# Autodesk Inventor assembly: SAFRS-L-0001
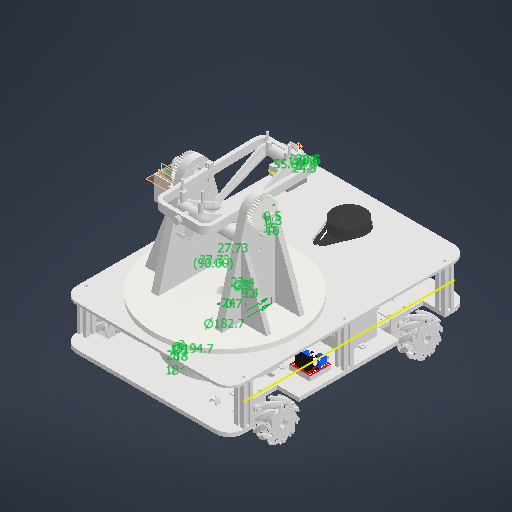
[picture p0: Inventor's stored thumbnail of the model, 512x512]
Saved by Autodesk Inventor 2026.2 (Build 302298000, 298)
## iProperties
Created: 2025-11-28
Part Number: SAFRS-L-0001
Document SubType Name: Assembly
Designer: jaewook
Author: jaewook
Title: SAFRS AGV Aseembly
## Documents named in this file (39)
- C:\Users\jk000\OneDrive\Desktop\git\SAFRS\mechanical\SAFRS_export\safrs_agv_assembly.iam
- C:\Users\jk000\OneDrive\Desktop\git\SAFRS\mechanical\SAFRS_export\01_parts\lower_plate.ipt
- C:\Users\jk000\OneDrive\Desktop\git\SAFRS\mechanical\SAFRS_export\01_parts\profile.ipt
- C:\Users\jk000\OneDrive\Desktop\git\SAFRS\mechanical\inventor\02_subassemblies\arduino_mega.iam
- C:\Users\jk000\OneDrive\Desktop\git\SAFRS\mechanical\inventor\02_subassemblies\stm32_assembly.iam
- C:\Users\jk000\OneDrive\Desktop\git\SAFRS\mechanical\inventor\02_subassemblies\L298N_motor_driver.iam
- C:\Users\jk000\OneDrive\Desktop\git\SAFRS\mechanical\SAFRS_export\01_parts\motor_connector.ipt
- C:\Users\jk000\OneDrive\Desktop\git\SAFRS\mechanical\SAFRS_export\01_parts\jgb37_520_motor_12v_319rpm.ipt
- C:\Users\jk000\OneDrive\Desktop\git\SAFRS\mechanical\inventor\02_subassemblies\dc_converter.iam
- C:\Users\jk000\OneDrive\Desktop\git\SAFRS\mechanical\SAFRS_export\01_parts\upper_plate.ipt
- C:\Users\jk000\OneDrive\Desktop\git\SAFRS\mechanical\inventor\02_subassemblies\yaw_motor_mount.iam
- C:\Users\jk000\OneDrive\Desktop\git\SAFRS\mechanical\SAFRS_export\01_parts\connector.ipt
- C:\Users\jk000\OneDrive\Desktop\git\SAFRS\mechanical\SAFRS_export\01_parts\carrier_v2.ipt
- C:\Users\jk000\OneDrive\Desktop\git\SAFRS\mechanical\SAFRS_export\01_parts\gear_support.ipt
- C:\Users\jk000\OneDrive\Desktop\git\SAFRS\mechanical\SAFRS_export\01_parts\spur_gear_15t.ipt
- C:\Users\jk000\OneDrive\Desktop\git\SAFRS\mechanical\SAFRS_export\01_parts\spur_gear_26t.ipt
- C:\Users\jk000\OneDrive\Desktop\git\SAFRS\mechanical\SAFRS_export\01_parts\spur_gear_13t.ipt
- C:\Users\jk000\OneDrive\Desktop\git\SAFRS\mechanical\SAFRS_export\01_parts\pitch_axis.ipt
- C:\Users\jk000\OneDrive\Desktop\git\SAFRS\mechanical\SAFRS_export\01_parts\pitch_axis_opposite.ipt
- C:\Users\jk000\OneDrive\Desktop\git\SAFRS\mechanical\SAFRS_export\01_parts\custom_bearing.ipt
- C:\Users\jk000\OneDrive\Desktop\git\SAFRS\mechanical\SAFRS_export\01_parts\spur_gear_22t.ipt
- C:\Users\jk000\OneDrive\Desktop\git\SAFRS\mechanical\SAFRS_export\01_parts\spur_gear_12t.ipt
- C:\Users\jk000\OneDrive\Desktop\git\SAFRS\mechanical\SAFRS_export\01_parts\pitch_motor.ipt
- C:\Users\jk000\OneDrive\Desktop\git\SAFRS\mechanical\inventor\02_subassemblies\roll_support_front_v2.iam
- C:\Users\jk000\OneDrive\Desktop\git\SAFRS\mechanical\inventor\02_subassemblies\roll_support_left_v1.iam
- C:\Users\jk000\OneDrive\Desktop\git\SAFRS\mechanical\inventor\02_subassemblies\roll_support_right.iam
- C:\Users\jk000\OneDrive\Desktop\git\SAFRS\mechanical\SAFRS_export\01_parts\key_v2.ipt
- C:\Users\jk000\OneDrive\Desktop\git\SAFRS\mechanical\SAFRS_export\01_parts\support_25mm.ipt
- C:\Users\jk000\OneDrive\Desktop\git\SAFRS\mechanical\inventor\02_subassemblies\fixer_assembly.iam
- C:\Users\jk000\OneDrive\Desktop\git\SAFRS\mechanical\SAFRS_export\01_parts\screw_v1.ipt
- C:\Users\jk000\OneDrive\Desktop\git\SAFRS\mechanical\inventor\02_subassemblies\lidar_base.iam
- C:\Users\jk000\OneDrive\Desktop\git\SAFRS\mechanical\SAFRS_export\01_parts\thrust_bearing_v1.ipt
- C:\Users\jk000\OneDrive\Desktop\git\SAFRS\mechanical\SAFRS_export\01_parts\short_screw.ipt
- C:\Users\jk000\OneDrive\Desktop\git\SAFRS\mechanical\SAFRS_export\01_parts\mecanum_wheel_75mm_left.ipt
- C:\Users\jk000\OneDrive\Desktop\git\SAFRS\mechanical\inventor\02_subassemblies\roll_support_rear_v1.iam
- C:\Users\jk000\OneDrive\Desktop\git\SAFRS\mechanical\inventor\02_subassemblies\battery_pack_mir.iam
- C:\Users\jk000\OneDrive\Desktop\git\SAFRS\mechanical\SAFRS_export\01_parts\pin.ipt
- C:\Users\jk000\OneDrive\Desktop\git\SAFRS\mechanical\SAFRS_export\01_parts\spur_gear_22t_opposite.ipt
- C:\Users\jk000\OneDrive\Desktop\git\SAFRS\mechanical\SAFRS_export\01_parts\Wire_aisle_v1.ipt
## Components (68 placed, 35 different names)
1. lower_plate:1 — 강체:1, 강체:2, 강체:3, 강체:4, 강체:5, 강체:6, 회전:1, 회전:2, 강체:8, 강체:9, 강체:10, 회전:3, 회전:4, 회전:5, 강체:11, 메이트:1, 메이트:2, 메이트:3, 메이트:6, 메이트:7, 메이트:9, 메이트:10, 메이트:18, 메이트:66, 메이트:67, 메이트:68, 메이트:69, 메이트:70, 메이트:71, 메이트:91, 메이트:92
2. profile:1 — 강체:1, 메이트:4
3. profile:2 — 강체:2
4. profile:3 — 강체:3, 메이트:5
5. profile:4 — 강체:4
6. profile:5 — 강체:5
7. profile:6 — 강체:6
8. arduino_mega:1 [sub-assembly] — 회전:1
9. stm32_assembly:1 [sub-assembly] — 회전:2
10. L298N_motor_driver:1 [sub-assembly] — 강체:8
11. L298N_motor_driver:2 [sub-assembly] — 강체:9
12. motor_connector:2 — 강체:10, 회전:9
13. motor_connector:3 — 회전:3, 회전:8
14. motor_connector:4 — 회전:4, 회전:7
15. motor_connector:5 — 회전:5, 회전:6
16. jgb37_520_motor_12v_319rpm:1 — 회전:6, 메이트:72, 메이트:73
17. jgb37_520_motor_12v_319rpm:2 — 회전:7, 메이트:74, 메이트:75
18. jgb37_520_motor_12v_319rpm:3 — 회전:8, 메이트:78, 메이트:79
19. jgb37_520_motor_12v_319rpm:4 — 회전:9, 메이트:76, 메이트:77
20. dc_converter:1 [sub-assembly] — 강체:11
21. dc_converter:2 [sub-assembly] — 메이트:1, 메이트:2, 메이트:3
22. upper_plate:1 — 메이트:4, 메이트:5, 메이트:89, 메이트:90, 메이트:93, 메이트:94, 메이트:95
23. yaw_motor_mount:1 [sub-assembly] — 메이트:6, 메이트:7, 메이트:8, 메이트:14
24. connector:1 — 메이트:8, 메이트:11, 메이트:12, 메이트:14, 메이트:15, 메이트:24
25. carrier_v2:1 — 메이트:9, 메이트:10, 메이트:18, 메이트:19, 메이트:20, 메이트:21, 메이트:22, 메이트:23, 플러쉬:1, 메이트:104, 메이트:105
26. gear_support:2 — 메이트:11, 메이트:12, 메이트:15, 메이트:16, 메이트:17
27. 스퍼 기어1:1 — 메이트:16, 메이트:17
28. 스퍼 기어2:1 — 메이트:19, 메이트:22
29. 스퍼 기어2:2 — 메이트:20, 메이트:23, 플러쉬:2
30. 스퍼 기어2:3 — 메이트:21, 플러쉬:1
31. 스퍼 기어1:2 — 메이트:24, 플러쉬:2, 메이트:25, 메이트:26, 메이트:27, 메이트:28, 메이트:29, 메이트:30
32. pitch_axis:1 — 메이트:25, 메이트:26, 메이트:27, 메이트:31, 메이트:32, 메이트:35, 메이트:37, 메이트:38, 메이트:44, 메이트:45
33. pitch_axis_opposite:1 — 메이트:28, 메이트:29, 메이트:30, 메이트:33, 메이트:34, 메이트:99
34. custom_bearing:1 — 메이트:31, 메이트:32, 메이트:36
35. custom_bearing:2 — 메이트:33, 메이트:34
36. 스퍼 기어2:4 — 메이트:35, 메이트:36, 메이트:59, 메이트:103
37. 스퍼 기어1:3 — 메이트:37, 메이트:38, 메이트:39, 메이트:40, 메이트:41
38. pitch_motor:1 — 메이트:39, 메이트:40, 메이트:41
39. pitch_motor:2 — 메이트:44, 메이트:45
40. roll_support_front_v2:1 [sub-assembly] — 메이트:52, 메이트:96, 강체:12
41. roll_support_rear_v1:1 [sub-assembly] — 메이트:97, 강체:13, 메이트:98, 메이트:100, 메이트:102
42. roll_support_left_v1:1 [sub-assembly] — 메이트:49, 메이트:50, 메이트:51
43. roll_support_right:1 [sub-assembly] — 메이트:49, 메이트:50, 메이트:51, 메이트:52
44. key_v2:1 — 메이트:59
45. support_25mm:1 — 메이트:60, 메이트:61, 메이트:66, 메이트:67
46. support_25mm:2 — 메이트:60, 메이트:61
47. support_25mm:3 — 메이트:62, 메이트:63, 메이트:68, 메이트:69
48. support_25mm:4 — 메이트:62, 메이트:63
49. support_25mm:5 — 메이트:64, 메이트:65, 메이트:70, 메이트:71
50. support_25mm:6 — 메이트:64, 메이트:65
51. fixer_assembly:1 [sub-assembly] — 메이트:89, 메이트:90
52. screw_v1:1 — 메이트:102, 메이트:103
53. lidar_base:1 [sub-assembly] — 메이트:93, 메이트:94, 메이트:95
54. thrust_bearing_v1:1
55. short_screw:1 — 메이트:72, 메이트:73, 메이트:80, 메이트:81
56. short_screw:2 — 메이트:74, 메이트:75, 메이트:82, 메이트:83
57. short_screw:3 — 메이트:76, 메이트:77, 메이트:86, 메이트:87
58. short_screw:4 — 메이트:78, 메이트:79, 메이트:84, 메이트:85
59. mecanum_wheel_75mm_left:1 — 메이트:80, 메이트:81
60. mecanum_wheel_75mm_left:2 — 메이트:82, 메이트:83
61. mecanum_wheel_75mm_left:3 — 메이트:84, 메이트:85
62. mecanum_wheel_75mm_left:4 — 메이트:86, 메이트:87
63. battery_pack_mir:1 [sub-assembly] — 메이트:91, 메이트:92
64. pin:1 — 메이트:96, 강체:12
65. pin:2 — 메이트:97, 강체:13
66. screw_v1:2 — 메이트:100, 메이트:101
67. spur_gear_22t_opposite:1 — 메이트:98, 메이트:99, 메이트:101
68. Wire_aisle_v1:1 — 메이트:104, 메이트:105
## Relationships (124: Mate 101, WeldJoint 12, RevoluteJoint 9, Flush 2)
- 강체:1 [WeldJoint]: lower_plate:1 ↔ profile:1
- 강체:2 [WeldJoint]: lower_plate:1 ↔ profile:2
- 강체:3 [WeldJoint]: lower_plate:1 ↔ profile:3
- 강체:4 [WeldJoint]: lower_plate:1 ↔ profile:4
- 강체:5 [WeldJoint]: lower_plate:1 ↔ profile:5
- 강체:6 [WeldJoint]: lower_plate:1 ↔ profile:6
- 회전:1 [RevoluteJoint]: lower_plate:1 ↔ arduino_mega:1
- 회전:2 [RevoluteJoint]: lower_plate:1 ↔ stm32_assembly:1
- 강체:8 [WeldJoint]: lower_plate:1 ↔ L298N_motor_driver:1
- 강체:9 [WeldJoint]: lower_plate:1 ↔ L298N_motor_driver:2
- 강체:10 [WeldJoint]: lower_plate:1 ↔ motor_connector:2
- 회전:3 [RevoluteJoint]: lower_plate:1 ↔ motor_connector:3
- 회전:4 [RevoluteJoint]: lower_plate:1 ↔ motor_connector:4
- 회전:5 [RevoluteJoint]: lower_plate:1 ↔ motor_connector:5
- 회전:6 [RevoluteJoint]: motor_connector:5 ↔ jgb37_520_motor_12v_319rpm:1
- 회전:7 [RevoluteJoint]: motor_connector:4 ↔ jgb37_520_motor_12v_319rpm:2
- 회전:8 [RevoluteJoint]: motor_connector:3 ↔ jgb37_520_motor_12v_319rpm:3
- 회전:9 [RevoluteJoint]: motor_connector:2 ↔ jgb37_520_motor_12v_319rpm:4
- 강체:11 [WeldJoint]: lower_plate:1 ↔ dc_converter:1
- 메이트:1 [Mate]: lower_plate:1 ↔ dc_converter:2
- 메이트:2 [Mate]: lower_plate:1 ↔ dc_converter:2
- 메이트:3 [Mate]: lower_plate:1 ↔ dc_converter:2
- 메이트:4 [Mate]: profile:1 ↔ upper_plate:1
- 메이트:5 [Mate]: profile:3 ↔ upper_plate:1
- 메이트:6 [Mate]: lower_plate:1 ↔ yaw_motor_mount:1
- 메이트:7 [Mate]: lower_plate:1 ↔ yaw_motor_mount:1
- 메이트:8 [Mate]: yaw_motor_mount:1 ↔ connector:1
- 메이트:9 [Mate]: lower_plate:1 ↔ carrier_v2:1
- 메이트:10 [Mate]: lower_plate:1 ↔ carrier_v2:1
- 메이트:11 [Mate]: connector:1 ↔ gear_support:2
- 메이트:12 [Mate]: connector:1 ↔ gear_support:2
- 메이트:14 [Mate]: yaw_motor_mount:1 ↔ connector:1
- 메이트:15 [Mate]: connector:1 ↔ gear_support:2
- 메이트:16 [Mate]: gear_support:2 ↔ 스퍼 기어1:1
- 메이트:17 [Mate]: gear_support:2 ↔ 스퍼 기어1:1
- 메이트:18 [Mate]: lower_plate:1 ↔ carrier_v2:1
- 메이트:19 [Mate]: carrier_v2:1 ↔ 스퍼 기어2:1
- 메이트:20 [Mate]: carrier_v2:1 ↔ 스퍼 기어2:2
- 메이트:21 [Mate]: carrier_v2:1 ↔ 스퍼 기어2:3
- 메이트:22 [Mate]: carrier_v2:1 ↔ 스퍼 기어2:1
- 메이트:23 [Mate]: carrier_v2:1 ↔ 스퍼 기어2:2
- 플러쉬:1 [Flush]: carrier_v2:1 ↔ 스퍼 기어2:3
- 메이트:24 [Mate]: connector:1 ↔ 스퍼 기어1:2
- 플러쉬:2 [Flush]: 스퍼 기어2:2 ↔ 스퍼 기어1:2
- 메이트:25 [Mate] (0.25 mm): 스퍼 기어1:2 ↔ pitch_axis:1
- 메이트:26 [Mate]: 스퍼 기어1:2 ↔ pitch_axis:1
- 메이트:27 [Mate]: 스퍼 기어1:2 ↔ pitch_axis:1
- 메이트:28 [Mate] (0.25 mm): 스퍼 기어1:2 ↔ pitch_axis_opposite:1
- 메이트:29 [Mate]: 스퍼 기어1:2 ↔ pitch_axis_opposite:1
- 메이트:30 [Mate]: 스퍼 기어1:2 ↔ pitch_axis_opposite:1
- 메이트:31 [Mate]: pitch_axis:1 ↔ custom_bearing:1
- 메이트:32 [Mate]: pitch_axis:1 ↔ custom_bearing:1
- 메이트:33 [Mate]: pitch_axis_opposite:1 ↔ custom_bearing:2
- 메이트:34 [Mate]: pitch_axis_opposite:1 ↔ custom_bearing:2
- 메이트:35 [Mate]: pitch_axis:1 ↔ 스퍼 기어2:4
- 메이트:36 [Mate]: custom_bearing:1 ↔ 스퍼 기어2:4
- 메이트:37 [Mate]: pitch_axis:1 ↔ 스퍼 기어1:3
- 메이트:38 [Mate]: pitch_axis:1 ↔ 스퍼 기어1:3
- 메이트:39 [Mate]: 스퍼 기어1:3 ↔ pitch_motor:1
- 메이트:40 [Mate]: 스퍼 기어1:3 ↔ pitch_motor:1
- 메이트:41 [Mate]: 스퍼 기어1:3 ↔ pitch_motor:1
- 메이트:44 [Mate]: pitch_axis:1 ↔ pitch_motor:2
- 메이트:45 [Mate]: pitch_axis:1 ↔ pitch_motor:2
- [Mate]: roll_support_front_v2:1 ↔ roll_support_rear_v1:1
- [Mate]: roll_support_front_v2:1 ↔ roll_support_rear_v1:1
- [Mate]: roll_support_front_v2:1 ↔ roll_support_rear_v1:1
- 메이트:49 [Mate]: roll_support_left_v1:1 ↔ roll_support_right:1
- 메이트:50 [Mate]: roll_support_left_v1:1 ↔ roll_support_right:1
- 메이트:51 [Mate]: roll_support_left_v1:1 ↔ roll_support_right:1
- 메이트:52 [Mate]: roll_support_front_v2:1 ↔ roll_support_right:1
- [Mate]: roll_support_rear_v1:1 ↔ roll_support_right:1
- [Mate]: custom_bearing:1 ↔ roll_support_rear_v1:1
- [Mate]: roll_support_rear_v1:1 ↔ key_v2:1
- [Mate]: roll_support_rear_v1:1 ↔ key_v2:1
- [Mate]: roll_support_rear_v1:1 ↔ key_v2:1
- [Mate]: pitch_axis:1 ↔ roll_support_rear_v1:1
- 메이트:59 [Mate]: 스퍼 기어2:4 ↔ key_v2:1
- 메이트:60 [Mate]: support_25mm:1 ↔ support_25mm:2
- 메이트:61 [Mate]: support_25mm:1 ↔ support_25mm:2
- 메이트:62 [Mate]: support_25mm:3 ↔ support_25mm:4
- 메이트:63 [Mate]: support_25mm:3 ↔ support_25mm:4
- 메이트:64 [Mate]: support_25mm:5 ↔ support_25mm:6
- 메이트:65 [Mate]: support_25mm:5 ↔ support_25mm:6
- 메이트:66 [Mate]: lower_plate:1 ↔ support_25mm:1
- 메이트:67 [Mate]: lower_plate:1 ↔ support_25mm:1
- 메이트:68 [Mate]: lower_plate:1 ↔ support_25mm:3
- 메이트:69 [Mate]: lower_plate:1 ↔ support_25mm:3
- 메이트:70 [Mate]: lower_plate:1 ↔ support_25mm:5
- 메이트:71 [Mate]: lower_plate:1 ↔ support_25mm:5
- 메이트:72 [Mate]: jgb37_520_motor_12v_319rpm:1 ↔ short_screw:1
- 메이트:73 [Mate]: jgb37_520_motor_12v_319rpm:1 ↔ short_screw:1
- 메이트:74 [Mate]: jgb37_520_motor_12v_319rpm:2 ↔ short_screw:2
- 메이트:75 [Mate]: jgb37_520_motor_12v_319rpm:2 ↔ short_screw:2
- 메이트:76 [Mate]: jgb37_520_motor_12v_319rpm:4 ↔ short_screw:3
- 메이트:77 [Mate]: jgb37_520_motor_12v_319rpm:4 ↔ short_screw:3
- 메이트:78 [Mate]: jgb37_520_motor_12v_319rpm:3 ↔ short_screw:4
- 메이트:79 [Mate]: jgb37_520_motor_12v_319rpm:3 ↔ short_screw:4
- 메이트:80 [Mate]: short_screw:1 ↔ mecanum_wheel_75mm_left:1
- 메이트:81 [Mate]: short_screw:1 ↔ mecanum_wheel_75mm_left:1
- 메이트:82 [Mate]: short_screw:2 ↔ mecanum_wheel_75mm_left:2
- 메이트:83 [Mate]: short_screw:2 ↔ mecanum_wheel_75mm_left:2
- 메이트:84 [Mate]: short_screw:4 ↔ mecanum_wheel_75mm_left:3
- 메이트:85 [Mate]: short_screw:4 ↔ mecanum_wheel_75mm_left:3
- 메이트:86 [Mate]: short_screw:3 ↔ mecanum_wheel_75mm_left:4
- 메이트:87 [Mate]: short_screw:3 ↔ mecanum_wheel_75mm_left:4
- 메이트:89 [Mate]: upper_plate:1 ↔ fixer_assembly:1
- 메이트:90 [Mate]: upper_plate:1 ↔ fixer_assembly:1
- 메이트:91 [Mate]: lower_plate:1 ↔ battery_pack_mir:1
- 메이트:92 [Mate]: lower_plate:1 ↔ battery_pack_mir:1
- 메이트:93 [Mate]: upper_plate:1 ↔ lidar_base:1
- 메이트:94 [Mate]: upper_plate:1 ↔ lidar_base:1
- 메이트:95 [Mate]: upper_plate:1 ↔ lidar_base:1
- 메이트:96 [Mate]: roll_support_front_v2:1 ↔ pin:1
- 강체:12 [WeldJoint]: roll_support_front_v2:1 ↔ pin:1
- 메이트:97 [Mate]: roll_support_rear_v1:1 ↔ pin:2
- 강체:13 [WeldJoint]: roll_support_rear_v1:1 ↔ pin:2
- 메이트:98 [Mate]: roll_support_rear_v1:1 ↔ spur_gear_22t_opposite:1
- 메이트:99 [Mate]: pitch_axis_opposite:1 ↔ spur_gear_22t_opposite:1
- 메이트:100 [Mate]: roll_support_rear_v1:1 ↔ screw_v1:2
- 메이트:101 [Mate]: screw_v1:2 ↔ spur_gear_22t_opposite:1
- 메이트:102 [Mate]: roll_support_rear_v1:1 ↔ screw_v1:1
- 메이트:103 [Mate]: 스퍼 기어2:4 ↔ screw_v1:1
- 메이트:104 [Mate]: carrier_v2:1 ↔ Wire_aisle_v1:1
- 메이트:105 [Mate]: carrier_v2:1 ↔ Wire_aisle_v1:1
